# Autodesk Inventor assembly: Steel-Lock-Steel
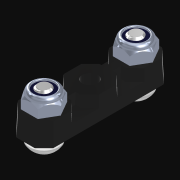
[picture p0: Inventor's stored thumbnail of the model, 180x180]
Saved by Autodesk Inventor 2021 (Build 250183000, 183)
## iProperties
Created: 2020-11-09
Part Number: Steel-Lock-Steel
Document SubType Name: Assembly
Designer: yuany
Author: yuany
## Documents named in this file (5)
- E:\VEX Cad\Library 1.2\Motion\Parts with Screws\Steel-Lock-Alu.iam
- E:\VEX Cad\Library 1.2\Motion\Bearing Flat.ipt
- E:\VEX Cad\Library 1.2\Structure\Hardware\Screw Steel - Hex\Screw 8-32 Steel .500.ipt
- E:\VEX Cad\Library 1.2\Structure\Hardware\Screw Steel - Hex.ipt
- E:\VEX Cad\Library 1.2\Structure\Hardware\Nut Thin Nylock.ipt
## Components (5 placed, 3 different names)
1. Bearing Flat:1 — Insert:4, Insert:6, Insert:7, Insert:8
2. Screw 8-32 Steel .500:1 — Insert:4
3. Nut Thin Nylock:2 — Insert:6
4. Screw 8-32 Steel .500:3 — Insert:8
5. Nut Thin Nylock:3 — Insert:7
## Relationships (4: Insert 4)
- Insert:4 (1.6002 mm): Bearing Flat:1 ↔ Screw 8-32 Steel .500:1
- Insert:6: Bearing Flat:1 ↔ Nut Thin Nylock:2
- Insert:7: Bearing Flat:1 ↔ Nut Thin Nylock:3
- Insert:8 (1.6002 mm): Bearing Flat:1 ↔ Screw 8-32 Steel .500:3
## Named parameters: Thickness = 1.6002 mm
